# Autodesk Inventor assembly: Lift - Bottom Motor Sprocket
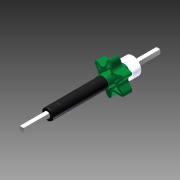
[picture p0: Inventor's stored thumbnail of the model, 180x180]
Saved by Autodesk Inventor 2012 (Build 160160000, 160)
## iProperties
Created: 2011-09-11
Part Number: Lift - Bottom Motor Sprocket
Document SubType Name: Assembly
Designer: Wade
Author: Wade
## Documents named in this file (6)
- C:\Users\Wade\Documents\1103 Robot - CAD Assembly\Lift - Bottom Motor Sprocket.iam
- C:\Users\Wade\Documents\24C VEX CAD Files\Drive Shafts\Drive Shaft (Square Bar) 4''.ipt
- C:\Users\Wade\Documents\24C VEX CAD Files\Gears & Pulleys\High Strength 6-Tooth Sprocket.ipt
- C:\Users\Wade\Documents\24C VEX CAD Files\Washers & Spacers\Spacer (Nylon), 0.250''.ipt
- C:\Users\Wade\Documents\24C VEX CAD Files\Washers & Spacers\Spacer (Thick), 8mm.ipt
- C:\Users\Wade\Documents\24C VEX CAD Files\Washers & Spacers\Spacer (Thin), 4.6mm.ipt
## Components (9 placed, 5 different names)
1. Drive Shaft (Square Bar) 4'':1 — Mate:3, Mate:4, Flush:2, Flush:3
2. High Strength 6-Tooth Sprocket:1 — Mate:3, Mate:4, Mate:5, Mate:6, Mate:11, Mate:12
3. Spacer (Nylon), 0.250'':1 — Mate:5, Mate:6, Flush:2
4. Spacer (Thick), 8mm:1 — Mate:14, Mate:15, Mate:16
5. Spacer (Thin), 4.6mm:1 — Mate:13, Mate:14
6. Spacer (Thick), 8mm:2 — Mate:11, Mate:12, Mate:13
7. Spacer (Thick), 8mm:3 — Mate:15, Mate:16, Mate:17, Mate:18
8. Spacer (Thick), 8mm:4 — Mate:17, Flush:3, Mate:19
9. Spacer (Thick), 8mm:5 — Mate:18, Mate:19
## Relationships (15: Mate 13, Flush 2)
- Mate:3: Drive Shaft (Square Bar) 4'':1 ↔ High Strength 6-Tooth Sprocket:1
- Mate:4: Drive Shaft (Square Bar) 4'':1 ↔ High Strength 6-Tooth Sprocket:1
- Mate:5: High Strength 6-Tooth Sprocket:1 ↔ Spacer (Nylon), 0.250'':1
- Mate:6: High Strength 6-Tooth Sprocket:1 ↔ Spacer (Nylon), 0.250'':1
- Mate:11: High Strength 6-Tooth Sprocket:1 ↔ Spacer (Thick), 8mm:2
- Mate:12: High Strength 6-Tooth Sprocket:1 ↔ Spacer (Thick), 8mm:2
- Mate:13: Spacer (Thin), 4.6mm:1 ↔ Spacer (Thick), 8mm:2
- Mate:14 (-1.27 mm): Spacer (Thick), 8mm:1 ↔ Spacer (Thin), 4.6mm:1
- Flush:2 (19.05 mm): Drive Shaft (Square Bar) 4'':1 ↔ Spacer (Nylon), 0.250'':1
- Mate:15 (-1.27 mm): Spacer (Thick), 8mm:1 ↔ Spacer (Thick), 8mm:3
- Mate:16: Spacer (Thick), 8mm:1 ↔ Spacer (Thick), 8mm:3
- Mate:17: Spacer (Thick), 8mm:3 ↔ Spacer (Thick), 8mm:4
- Flush:3 (19.05 mm): Drive Shaft (Square Bar) 4'':1 ↔ Spacer (Thick), 8mm:4
- Mate:18: Spacer (Thick), 8mm:3 ↔ Spacer (Thick), 8mm:5
- Mate:19: Spacer (Thick), 8mm:4 ↔ Spacer (Thick), 8mm:5
